# Autodesk Inventor assembly: 总装
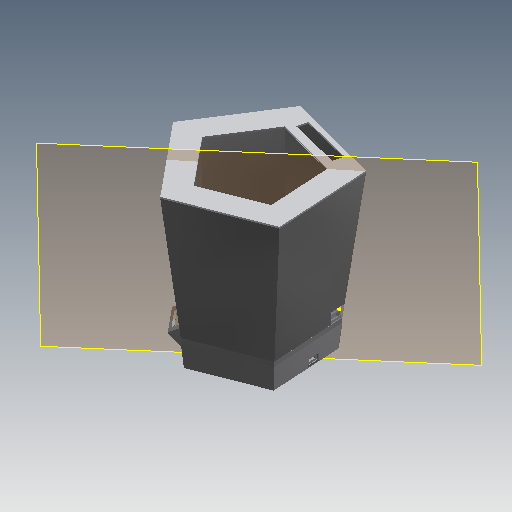
[picture p0: Inventor's stored thumbnail of the model, 512x512]
Saved by Autodesk Inventor 2018 (Build 220112000, 112)
## iProperties
Created: 2021-03-07
Part Number: 总装
Material: 常规
Document SubType Name: Assembly
Designer: OHHHHHHHHHH
Author: OHHHHHHHHHH
## Documents named in this file (8)
- C:\Users\OHHHHHHHHHH\Desktop\浇花系统三代\总装.iam
- C:\Users\OHHHHHHHHHH\Desktop\浇花系统第二代\鸦片.ipt
- C:\Users\OHHHHHHHHHH\Desktop\浇花系统第二代\压片下.ipt
- C:\Users\OHHHHHHHHHH\Desktop\浇花系统第二代\磁铁.ipt
- C:\Users\OHHHHHHHHHH\Desktop\浇花系统三代\花盆底座.ipt
- C:\Users\OHHHHHHHHHH\Desktop\浇花系统三代\花盆主体.ipt
- C:\Users\OHHHHHHHHHH\Desktop\浇花系统第二代\花盆主体拼接.ipt
- C:\Users\OHHHHHHHHHH\Desktop\浇花系统三代\端盖.ipt
## Components (8 placed, 7 different names)
1. 鸦片:1 — 配合:1, 配合:2, 表面齐平:1, 配合:9, 配合:10
2. 压片下:1 — 配合:1, 配合:2, 配合:3, 配合:4, 配合:6, 表面齐平:1
3. 磁铁:1 — 配合:3, 配合:5, 配合:6
4. 花盆底座:1 — 配合:7, 配合:8, 角度:1, 配合:16
5. 磁铁:2 — 配合:4, 配合:5
6. 花盆主体:1 — 配合:7, 配合:8, 配合:9, 配合:10, 角度:1, 配合:11, 配合:12, 配合:13, 表面齐平:2, 表面齐平:3, 配合:14
7. 花盆主体拼接:1 — 配合:11, 配合:12, 配合:13
8. 端盖:1 — 表面齐平:2, 表面齐平:3, 配合:14, 配合:15, 配合:17
## Relationships (21: Mate 17, Flush 3, Angle 1)
- 配合:1 [Mate]: 鸦片:1 ↔ 压片下:1
- 配合:2 [Mate]: 鸦片:1 ↔ 压片下:1
- 配合:3 [Mate]: 压片下:1 ↔ 磁铁:1
- 配合:4 [Mate]: 压片下:1 ↔ 磁铁:2
- 配合:5 [Mate]: 磁铁:1 ↔ 磁铁:2
- 配合:6 [Mate]: 压片下:1 ↔ 磁铁:1
- 表面齐平:1 [Flush]: 鸦片:1 ↔ 压片下:1
- 配合:7 [Mate]: 花盆底座:1 ↔ 花盆主体:1
- 配合:8 [Mate]: 花盆底座:1 ↔ 花盆主体:1
- 配合:9 [Mate]: 鸦片:1 ↔ 花盆主体:1
- 配合:10 [Mate]: 鸦片:1 ↔ 花盆主体:1
- 角度:1 [Angle] (0 deg): 花盆底座:1 ↔ 花盆主体:1
- 配合:11 [Mate]: 花盆主体:1 ↔ 花盆主体拼接:1
- 配合:12 [Mate]: 花盆主体:1 ↔ 花盆主体拼接:1
- 配合:13 [Mate]: 花盆主体:1 ↔ 花盆主体拼接:1
- 表面齐平:2 [Flush]: 花盆主体:1 ↔ 端盖:1
- 表面齐平:3 [Flush]: 花盆主体:1 ↔ 端盖:1
- 配合:14 [Mate]: 花盆主体:1 ↔ 端盖:1
- 配合:15 [Mate]: 端盖:1
- 配合:16 [Mate]: 花盆底座:1
- 配合:17 [Mate]: 端盖:1
